# Autodesk Inventor assembly: backplane
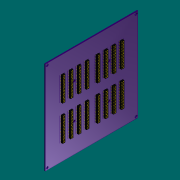
[picture p0: Inventor's stored thumbnail of the model, 180x180]
Saved by Autodesk Inventor 2016 (Build 200138000, 138)
## iProperties
Created: 2015-12-22
Part Number: backplane
Description: for SolidWorks
Document SubType Name: Assembly
Designer: sawai
Authority: Unknown
Sending System: Diptrace
Preprocessor: Open CASCADE STEP processor 6.6
Title: C:\Users\sawai\Desktop\backplane.step
Author: sawai
## Documents named in this file (4)
- C:\Users\sawaiz\oneDrive\projects\modularRICHBackplane\cad\backplane.iam
- C:\Users\sawaiz\oneDrive\projects\modularRICHBackplane\cad\backplane.ipt
- C:\Users\sawaiz\oneDrive\projects\modularRICHBackplane\cad\connectors\N182GFNS-RC.ipt
- C:\Users\sawaiz\oneDrive\projects\modularRICHBackplane\cad\connectors\2x16header.ipt
## Components (33 placed, 3 different names)
1. backplane:1 — Mate:2, Angle:2, Mate:3, Angle:3
2. N182GFNS-RC:17 — Mate:2, Angle:2
3. N182GFNS-RC:18
4. N182GFNS-RC:19
5. N182GFNS-RC:20
6. N182GFNS-RC:21
7. N182GFNS-RC:22
8. N182GFNS-RC:23
9. N182GFNS-RC:24
10. N182GFNS-RC:25
11. N182GFNS-RC:26
12. N182GFNS-RC:27
13. N182GFNS-RC:28
14. N182GFNS-RC:29
15. N182GFNS-RC:30
16. N182GFNS-RC:31
17. N182GFNS-RC:32
18. 2x16header:1 — Mate:3, Angle:3
19. 2x16header:2
20. 2x16header:3
21. 2x16header:4
22. 2x16header:5
23. 2x16header:6
24. 2x16header:7
25. 2x16header:8
26. 2x16header:9
27. 2x16header:10
28. 2x16header:11
29. 2x16header:12
30. 2x16header:13
31. 2x16header:14
32. 2x16header:15
33. 2x16header:16
## Component patterns: (4 elements), (4 elements), (4 elements, first: N182GFNS-RC:17), Component Pattern 5:2 (4 elements), Component Pattern 5:3 (4 elements), Component Pattern 5:4 (4 elements), (4 elements, first: 2x16header:1), Component Pattern 7:2 (4 elements), Component Pattern 7:3 (4 elements), Component Pattern 7:4 (4 elements)
## Relationships (4: Mate 2, Angle 2)
- Mate:2: backplane:1 ↔ N182GFNS-RC:17
- Angle:2 (0 deg): backplane:1 ↔ N182GFNS-RC:17
- Mate:3: backplane:1 ↔ 2x16header:1
- Angle:3 (0 deg): backplane:1 ↔ 2x16header:1
